# Autodesk Inventor assembly: PIP-Boy 6400 Mk_I Computer Subassembly
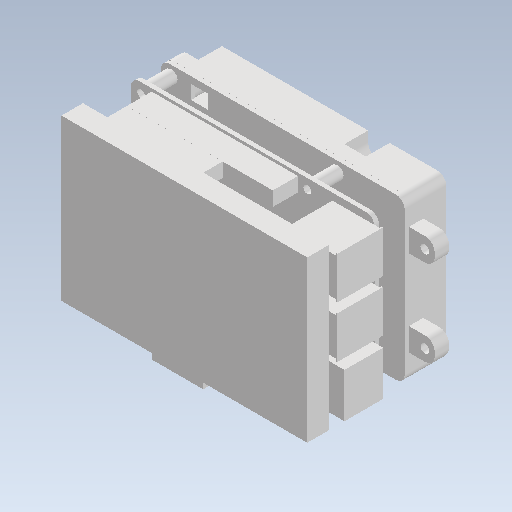
[picture p0: Inventor's stored thumbnail of the model, 512x512]
Saved by Autodesk Inventor 2021 (Build 250183000, 183)
## iProperties
Created: 2021-04-19
Part Number: PIP-Boy 6400 Mk_I Computer Subassembly
Document SubType Name: Assembly
Designer: trent
Author: trent
## Documents named in this file (7)
- C:\Users\EmeraldLeeTiger\OneDrive - wmpenn.edu\Personal\PIP-Boy 6400 Mk.I\PIP-Boy 6400 Mk_I Computer Subassembly.iam
- C:\Users\EmeraldLeeTiger\OneDrive - wmpenn.edu\Personal\PIP-Boy 6400 Mk.I\RaspberryPi3 Computer_Standoff.ipt
- C:\Users\EmeraldLeeTiger\OneDrive - wmpenn.edu\Personal\PIP-Boy 6400 Mk.I\RaspberryPi3 Computer_Battery Board.ipt
- C:\Users\EmeraldLeeTiger\OneDrive - wmpenn.edu\Personal\PIP-Boy 6400 Mk.I\RaspberryPi3 Computer_Pi Board.ipt
- C:\Users\EmeraldLeeTiger\OneDrive - wmpenn.edu\Personal\PIP-Boy 6400 Mk.I\RaspberryPi3 Comupter_HDMI Jumper.ipt
- C:\Users\EmeraldLeeTiger\OneDrive - wmpenn.edu\Personal\PIP-Boy 6400 Mk.I\RaspberryPi3 Computer_Screen.ipt
- C:\Users\EmeraldLeeTiger\OneDrive - wmpenn.edu\Personal\PIP-Boy 6400 Mk.I\RaspberryPi3 Computer_Mounting Bracket.ipt
## Components (9 placed, 6 different names)
1. RaspberryPi3 Computer_Standoff:1 — Mate:14, Mate:17
2. RaspberryPi3 Computer_Standoff:2
3. RaspberryPi3 Computer_Standoff:3
4. RaspberryPi3 Computer_Standoff:4 — Mate:12, Mate:13, Mate:15, Mate:16
5. RaspberryPi3 Computer_Battery Board:1 — Mate:12, Mate:13, Mate:14, Mate:23, Mate:24, Mate:25
6. RaspberryPi3 Computer_Pi Board:1 — Mate:15, Mate:16, Mate:17, Mate:21, Flush:1, Flush:2
7. RaspberryPi3 Comupter_HDMI Jumper:1 — Mate:22, Flush:3, Flush:4
8. RaspberryPi3 Computer_Screen:1 — Mate:21, Flush:1, Flush:2, Mate:22, Flush:3, Flush:4
9. RaspberryPi3 Computer_Mounting Bracket:1 — Mate:23, Mate:24, Mate:25
## Relationships (15: Mate 11, Flush 4)
- Mate:12: RaspberryPi3 Computer_Standoff:4 ↔ RaspberryPi3 Computer_Battery Board:1
- Mate:13: RaspberryPi3 Computer_Standoff:4 ↔ RaspberryPi3 Computer_Battery Board:1
- Mate:14: RaspberryPi3 Computer_Standoff:1 ↔ RaspberryPi3 Computer_Battery Board:1
- Mate:15: RaspberryPi3 Computer_Standoff:4 ↔ RaspberryPi3 Computer_Pi Board:1
- Mate:16: RaspberryPi3 Computer_Standoff:4 ↔ RaspberryPi3 Computer_Pi Board:1
- Mate:17: RaspberryPi3 Computer_Standoff:1 ↔ RaspberryPi3 Computer_Pi Board:1
- Mate:21: RaspberryPi3 Computer_Pi Board:1 ↔ RaspberryPi3 Computer_Screen:1
- Flush:1: RaspberryPi3 Computer_Pi Board:1 ↔ RaspberryPi3 Computer_Screen:1
- Flush:2: RaspberryPi3 Computer_Pi Board:1 ↔ RaspberryPi3 Computer_Screen:1
- Mate:22: RaspberryPi3 Comupter_HDMI Jumper:1 ↔ RaspberryPi3 Computer_Screen:1
- Flush:3 (0.254 mm): RaspberryPi3 Comupter_HDMI Jumper:1 ↔ RaspberryPi3 Computer_Screen:1
- Flush:4 (1.016 mm): RaspberryPi3 Comupter_HDMI Jumper:1 ↔ RaspberryPi3 Computer_Screen:1
- Mate:23: RaspberryPi3 Computer_Battery Board:1 ↔ RaspberryPi3 Computer_Mounting Bracket:1
- Mate:24: RaspberryPi3 Computer_Battery Board:1 ↔ RaspberryPi3 Computer_Mounting Bracket:1
- Mate:25: RaspberryPi3 Computer_Battery Board:1 ↔ RaspberryPi3 Computer_Mounting Bracket:1
